# Autodesk Inventor assembly: Cylinder Piston Rod
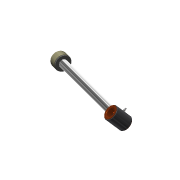
[picture p0: Inventor's stored thumbnail of the model, 180x180]
Saved by Autodesk Inventor 2022 Beta2 (Build 260130000, 130) ContinuousBuild 0
## iProperties
Shininess: 20.0
Length Units: 11269
Angle Units: 11279
Time Units: 11290
Mass Units: 11283
Length Display Precision: 3
Angle Display Precision: 2
Created: 2001-06-29
Part Number: Cylinder Piston Rod
Description: Piston rod compl. 63/32-350
Document SubType Name: Assembly
Designer: Joe M
Engineer: Joe M
Density: 0.0
Volumn: 0.0
Area: 0.0
PropertySet Name: Model Information
Control State: 0
Master: False
Checked Out: False
Title: Kolvstång kompl. 63/32-350
Author: Joe M
## Documents named in this file (6)
- C:\Autodesk Inventor 2021 Intro Practice Files\BOM\Cylinder Piston Rod.iam
- C:\Autodesk Inventor 2021 Intro Practice Files\BOM\3136 1144 60.ipt
- C:\Autodesk Inventor 2021 Intro Practice Files\BOM\3136 7048 80.ipt
- C:\Autodesk Inventor 2021 Intro Practice Files\BOM\0544 1100 09.ipt
- C:\Autodesk Inventor 2021 Intro Practice Files\BOM\3136 1117 73.ipt
- C:\Autodesk Inventor 2021 Intro Practice Files\BOM\3136 7009 52.ipt
## Components (6 placed, 5 different names)
1. 3136 1144 60:1 — Insert:1, Mate:1, Mate:2, Insert:2, Mate:3, Flush:1
2. 3136 7048 80:1 — Insert:1
3. 3136 7048 80:2 — Insert:2
4. 0544 1100 09:1 — Mate:1, Mate:2
5. 3136 1117 73:1 — Mate:3, Flush:1, Mate:4, Mate:5
6. 3136 7009 52:1 — Mate:4, Mate:5
## Relationships (8: Mate 5, Insert 2, Flush 1)
- Insert:1: 3136 1144 60:1 ↔ 3136 7048 80:1
- Mate:1: 3136 1144 60:1 ↔ 0544 1100 09:1
- Mate:2 (30 mm): 3136 1144 60:1 ↔ 0544 1100 09:1
- Insert:2: 3136 1144 60:1 ↔ 3136 7048 80:2
- Mate:3: 3136 1144 60:1 ↔ 3136 1117 73:1
- Flush:1: 3136 1144 60:1 ↔ 3136 1117 73:1
- Mate:4: 3136 1117 73:1 ↔ 3136 7009 52:1
- Mate:5: 3136 1117 73:1 ↔ 3136 7009 52:1
## Named parameters: d0_d3 = 0 mm, d1_d4 = 0 mm, d2_d5 = 30 mm, d3_d6 = 0 mm, d4_d12 = 0 mm, d5_d13 = 0 mm, d6_d14 = 0 mm, d7_d15 = 0 mm
